# Autodesk Inventor assembly: bottomCNC
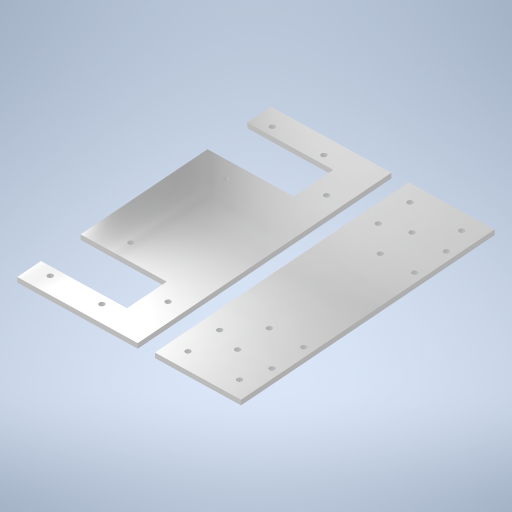
[picture p0: Inventor's stored thumbnail of the model, 512x512]
Saved by Autodesk Inventor 2024 (Build 280153000, 153)
## iProperties
Created: 2023-10-26
Part Number: bottomCNC
Document SubType Name: Assembly
Designer: jwith
Author: jwith
## Documents named in this file (3)
- C:\Users\jwith\OneDrive\kikaiken\inventor\general-useLandRobotV1\bottomCNC.iam
- C:\Users\jwith\OneDrive\kikaiken\inventor\general-useLandRobotV1\frontPlate.ipt
- C:\Users\jwith\OneDrive\kikaiken\inventor\general-useLandRobotV1\backPlate.ipt
## Components (2 placed, 2 different names)
1. frontPlate:1 — フラッシュ:1, メイト:1, フラッシュ:3
2. backPlate:1 — フラッシュ:2, メイト:1, フラッシュ:3
## Relationships (4: Flush 3, Mate 1)
- フラッシュ:1 [Flush]: frontPlate:1
- フラッシュ:2 [Flush]: backPlate:1
- メイト:1 [Mate] (10 mm): frontPlate:1 ↔ backPlate:1
- フラッシュ:3 [Flush]: frontPlate:1 ↔ backPlate:1
